# Autodesk Inventor assembly: Extruder 2.3
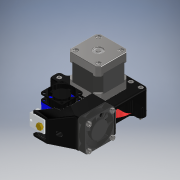
[picture p0: Inventor's stored thumbnail of the model, 180x180]
Saved by Autodesk Inventor 2020.2 (Build 242310000, 310)
## iProperties
Created: 2020-03-20
Part Number: Extruder 2.3
Document SubType Name: Assembly
Designer: rah75
Author: rah75
## Documents named in this file (30)
- C:\Users\rah75\Box\CAD\3D Printer\X Carriage\Extruder 2.3.iam
- C:\Users\rah75\Box\CAD\3D Printer\X Carriage\Lower Extruder Block.ipt
- C:\Users\rah75\Box\CAD\3D Printer\X Carriage\Extruder Motor Plate 2.ipt
- C:\Users\rah75\Box\CAD\3D Printer\X Carriage\Extruder Clamp Block.ipt
- C:\Users\rah75\Box\CAD\3D Printer\X Carriage\x carraige plate new blocked.ipt
- C:\Users\rah75\Box\CAD\3D Printer\X Carriage\Extruder Mount Plate 2.ipt
- C:\Users\rah75\Box\CAD\3D Printer\X Carriage\Extruder Plate.ipt
- C:\Users\rah75\Box\CAD\Stock Components\Motors\NEMA 17 Shorted Shaft.ipt
- C:\Users\rah75\Box\CAD\3D Printer\X Carriage\Drive Gear 0.8m57t Internal.ipt
- C:\Users\rah75\Box\CAD\Stock Components\Power Transmission\Bearings\5x16mm_625-2z.ipt
- C:\Users\rah75\Box\CAD\Stock Components\Power Transmission\Extruder Knob.ipt
- C:\Users\rah75\Box\CAD\3D Printer\X Carriage\Fillament Guide.ipt
- C:\Users\rah75\Box\CAD\3D Printer\e3d-v6-hotend-3\e3d v6.iam
- C:\Users\rah75\Box\CAD\3D Printer\X Carriage\Drive Pinion 0.8m12t 2.ipt
- C:\Users\rah75\Box\CAD\3D Printer\X Carriage\Drive Shaft.ipt
- C:\Users\rah75\Box\CAD\3D Printer\X Carriage\Idler Shaft.ipt
- C:\Users\rah75\Box\CAD\Stock Components\Fasteners\Screws\SHCS M3x20.ipt
- C:\Users\rah75\Box\CAD\Stock Components\Fasteners\Screws\SHCS M3x35.ipt
- C:\Users\rah75\Box\CAD\Stock Components\Electrical\Inductive Sensor 18mmx70mm.ipt
- C:\Users\rah75\Box\CAD\3D Printer\X Carriage\Inductive Sensor Mount.ipt
- C:\Users\rah75\Box\CAD\Stock Components\Electrical\40x40mm Fan.ipt
- C:\Users\rah75\Box\CAD\3D Printer\X Carriage\Fan Duct.ipt
- C:\Users\rah75\Box\CAD\Stock Components\Fasteners\Nuts\M3 Heat Set Inserts.ipt
- C:\Users\rah75\Box\CAD\Stock Components\Fasteners\Screws\SHCS M3x8.ipt
- C:\Users\rah75\Box\CAD\Stock Components\Fasteners\Screws\SHCS M3x10.ipt
- C:\Users\rah75\Box\CAD\Stock Components\Fasteners\Screws\SHCS M3x30.ipt
- C:\Users\rah75\Box\CAD\Stock Components\Fasteners\Screws\SHCS M3x12.ipt
- C:\Users\rah75\Box\CAD\Stock Components\Fasteners\Nuts\M3 Nut.ipt
- C:\Users\rah75\Box\CAD\Stock Components\Fasteners\Screws\Set Screws\Set Screw M3x6.ipt
- C:\Users\rah75\Box\CAD\Stock Components\Fasteners\Screws\SHCS M3x5.ipt
## Components (51 placed, 29 different names)
1. Lower Extruder Block:2 — Mate:3, Mate:4, Insert:3, Insert:5, Mate:9, Mate:10, Angle:1, Insert:11, Mate:21, Flush:4, Insert:20, Insert:25
2. Extruder Motor Plate 2:2 — Mate:4, Insert:3, Insert:4, Mate:5, Mate:6, Mate:8, Insert:6, Mate:11, Insert:16, Insert:17, Insert:18, Insert:19, Angle:3, Insert:23, Insert:24, Insert:28, Insert:29, Insert:41, Insert:42
3. Extruder Clamp Block:1 — Insert:4, Mate:5, Insert:7, Mate:13, Mate:15, Angle:2, Mate:19, Insert:14, Insert:15, Insert:21, Insert:22, Insert:39, Insert:40
4. x carraige plate new blocked:1 — Mate:3, Mate:7, Mate:8
5. Extruder Mount Plate 2:1 — Insert:5, Mate:6, Mate:7, Insert:8, Insert:30, Insert:31
6. Extruder Plate:1 — Mate:9, Mate:10, Angle:1, Mate:20, Mate:25
7. NEMA 17 Shorted Shaft:1 — Insert:6, Mate:11, Mate:18, Flush:1, Angle:4, Angle:5
8. Drive Gear 0.8m57t Internal:1 — Insert:9, Insert:10, Insert:37, Mate:28, Insert:43
9. Extruder Knob:1 — Insert:10, Mate:12, Mate:16
10. Fillament Guide:1 — Mate:15, Mate:16, Mate:17, Angle:2
11. e3d v6:1 [sub-assembly] — Insert:11, Angle:5
12. Drive Pinion 0.8m12t 2:1 — Mate:18, Flush:1
13. Drive Shaft:1 — Insert:12
14. Idler Shaft:1 — Insert:13
15. Inductive Sensor 18mmx70mm:1 — Angle:3, Mate:22
16. Inductive Sensor Mount:1 — Mate:20, Mate:21, Angle:4, Mate:22, Insert:26
17. 40x40mm Fan:1 — Insert:32, Mate:26, Insert:33, Insert:34, Insert:35, Insert:36
18. Fan Duct:1 — Flush:4, Mate:25, Insert:27, Insert:32, Mate:26
19. 5x16mm_625-2z:2 — Insert:8, Insert:9
20. 5x16mm_625-2z:3 — Mate:12, Mate:13, Mate:17, Mate:19, Insert:13
21. 5x16mm_625-2z:1 — Insert:7, Insert:12
22. M3 Nut:3 — Insert:40
23. M3 Nut:4 — Insert:39
24. SHCS M3x5:1 — Insert:42
25. SHCS M3x5:2 — Insert:41
26. M3 Heat Set Inserts:1 — Insert:20, Mate:27
27. M3 Heat Set Inserts:2 — Insert:22
28. M3 Heat Set Inserts:3 — Insert:21
29. SHCS M3x8:1 — Insert:23
30. SHCS M3x8:2 — Insert:24
31. M3 Heat Set Inserts:4 — Insert:25
32. SHCS M3x10:1 — Insert:26
33. SHCS M3x10:2 — Insert:27, Mate:27
34. M3 Heat Set Inserts:5 — Insert:28
35. M3 Heat Set Inserts:6 — Insert:29
36. SHCS M3x30:1 — Insert:30
37. SHCS M3x30:2 — Insert:31
38. SHCS M3x12:1 — Insert:33
39. SHCS M3x12:2 — Insert:34
40. SHCS M3x12:3 — Insert:35
41. SHCS M3x12:4 — Insert:36
42. M3 Nut:1 — Insert:37, Flush:6
43. M3 Nut:2 — Insert:43, Mate:29, Flush:5
44. Set Screw M3x6:1 — Mate:28, Flush:6
45. Set Screw M3x6:2 — Mate:29, Flush:5
46. SHCS M3x20:2 — Insert:14
47. SHCS M3x35:1 — Insert:18
48. SHCS M3x35:2 — Insert:17
49. SHCS M3x35:3 — Insert:16
50. SHCS M3x35:4 — Insert:19
51. SHCS M3x20:1 — Insert:15
## Relationships (73: Insert 40, Mate 24, Angle 5, Flush 4)
- Mate:3: Lower Extruder Block:2 ↔ x carraige plate new blocked:1
- Mate:4: Lower Extruder Block:2 ↔ Extruder Motor Plate 2:2
- Insert:3: Lower Extruder Block:2 ↔ Extruder Motor Plate 2:2
- Insert:4: Extruder Motor Plate 2:2 ↔ Extruder Clamp Block:1
- Mate:5: Extruder Motor Plate 2:2 ↔ Extruder Clamp Block:1
- Insert:5: Lower Extruder Block:2 ↔ Extruder Mount Plate 2:1
- Mate:6: Extruder Motor Plate 2:2 ↔ Extruder Mount Plate 2:1
- Mate:7: x carraige plate new blocked:1 ↔ Extruder Mount Plate 2:1
- Mate:8: Extruder Motor Plate 2:2 ↔ x carraige plate new blocked:1
- Mate:9: Lower Extruder Block:2 ↔ Extruder Plate:1
- Mate:10: Lower Extruder Block:2 ↔ Extruder Plate:1
- Angle:1 (0 deg): Lower Extruder Block:2 ↔ Extruder Plate:1
- Insert:6: Extruder Motor Plate 2:2 ↔ NEMA 17 Shorted Shaft:1
- Mate:11: Extruder Motor Plate 2:2 ↔ NEMA 17 Shorted Shaft:1
- Insert:7: Extruder Clamp Block:1 ↔ 5x16mm_625-2z:1
- Insert:8: Extruder Mount Plate 2:1 ↔ 5x16mm_625-2z:2
- Insert:9 (0.5 mm): Drive Gear 0.8m57t Internal:1 ↔ 5x16mm_625-2z:2
- Insert:10 (1.5 mm): Drive Gear 0.8m57t Internal:1 ↔ Extruder Knob:1
- Mate:12: Extruder Knob:1 ↔ 5x16mm_625-2z:3
- Mate:13 (0.25 mm): Extruder Clamp Block:1 ↔ 5x16mm_625-2z:3
- Mate:15: Extruder Clamp Block:1 ↔ Fillament Guide:1
- Mate:16: Extruder Knob:1 ↔ Fillament Guide:1
- Mate:17: Fillament Guide:1 ↔ 5x16mm_625-2z:3
- Angle:2 (0 deg): Extruder Clamp Block:1 ↔ Fillament Guide:1
- Insert:11: Lower Extruder Block:2 ↔ e3d v6:1
- Mate:18: NEMA 17 Shorted Shaft:1 ↔ Drive Pinion 0.8m12t 2:1
- Flush:1 (-0.75 mm): NEMA 17 Shorted Shaft:1 ↔ Drive Pinion 0.8m12t 2:1
- Insert:12: Drive Shaft:1 ↔ 5x16mm_625-2z:1
- Mate:19: Extruder Clamp Block:1 ↔ 5x16mm_625-2z:3
- Insert:13 (-4.5 mm): Idler Shaft:1 ↔ 5x16mm_625-2z:3
- Insert:14 (3 mm): Extruder Clamp Block:1 ↔ SHCS M3x20:2
- Insert:15 (3 mm): Extruder Clamp Block:1 ↔ SHCS M3x20:1
- Insert:16: Extruder Motor Plate 2:2 ↔ SHCS M3x35:3
- Insert:17: Extruder Motor Plate 2:2 ↔ SHCS M3x35:2
- Insert:18: Extruder Motor Plate 2:2 ↔ SHCS M3x35:1
- Insert:19: Extruder Motor Plate 2:2 ↔ SHCS M3x35:4
- Angle:3 (0 deg): Extruder Motor Plate 2:2 ↔ Inductive Sensor 18mmx70mm:1
- Mate:20: Extruder Plate:1 ↔ Inductive Sensor Mount:1
- Mate:21: Lower Extruder Block:2 ↔ Inductive Sensor Mount:1
- Angle:4 (180 deg): NEMA 17 Shorted Shaft:1 ↔ Inductive Sensor Mount:1
- Mate:22: Inductive Sensor 18mmx70mm:1 ↔ Inductive Sensor Mount:1
- Angle:5 (0 deg): NEMA 17 Shorted Shaft:1 ↔ e3d v6:1
- Flush:4: Lower Extruder Block:2 ↔ Fan Duct:1
- Mate:25: Extruder Plate:1 ↔ Fan Duct:1
- Insert:20: Lower Extruder Block:2 ↔ M3 Heat Set Inserts:1
- Insert:21: Extruder Clamp Block:1 ↔ M3 Heat Set Inserts:3
- Insert:22: Extruder Clamp Block:1 ↔ M3 Heat Set Inserts:2
- Insert:23: Extruder Motor Plate 2:2 ↔ SHCS M3x8:1
- Insert:24: Extruder Motor Plate 2:2 ↔ SHCS M3x8:2
- Insert:25: Lower Extruder Block:2 ↔ M3 Heat Set Inserts:4
- Insert:26 (-4 mm): Inductive Sensor Mount:1 ↔ SHCS M3x10:1
- Insert:27: Fan Duct:1 ↔ SHCS M3x10:2
- Insert:28: Extruder Motor Plate 2:2 ↔ M3 Heat Set Inserts:5
- Insert:29: Extruder Motor Plate 2:2 ↔ M3 Heat Set Inserts:6
- Insert:30: Extruder Mount Plate 2:1 ↔ SHCS M3x30:1
- Insert:31: Extruder Mount Plate 2:1 ↔ SHCS M3x30:2
- Insert:32: 40x40mm Fan:1 ↔ Fan Duct:1
- Mate:26: 40x40mm Fan:1 ↔ Fan Duct:1
- Mate:27: M3 Heat Set Inserts:1 ↔ SHCS M3x10:2
- Insert:33: 40x40mm Fan:1 ↔ SHCS M3x12:1
- Insert:34: 40x40mm Fan:1 ↔ SHCS M3x12:2
- Insert:35: 40x40mm Fan:1 ↔ SHCS M3x12:3
- Insert:36: 40x40mm Fan:1 ↔ SHCS M3x12:4
- Insert:37: Drive Gear 0.8m57t Internal:1 ↔ M3 Nut:1
- Mate:28: Drive Gear 0.8m57t Internal:1 ↔ Set Screw M3x6:1
- Insert:39: Extruder Clamp Block:1 ↔ M3 Nut:4
- Insert:40: Extruder Clamp Block:1 ↔ M3 Nut:3
- Insert:41: Extruder Motor Plate 2:2 ↔ SHCS M3x5:2
- Insert:42: Extruder Motor Plate 2:2 ↔ SHCS M3x5:1
- Insert:43: Drive Gear 0.8m57t Internal:1 ↔ M3 Nut:2
- Mate:29: M3 Nut:2 ↔ Set Screw M3x6:2
- Flush:5 (2.5 mm): M3 Nut:2 ↔ Set Screw M3x6:2
- Flush:6 (2.5 mm): M3 Nut:1 ↔ Set Screw M3x6:1
